# Autodesk Inventor assembly: 三組合窗_MIR2
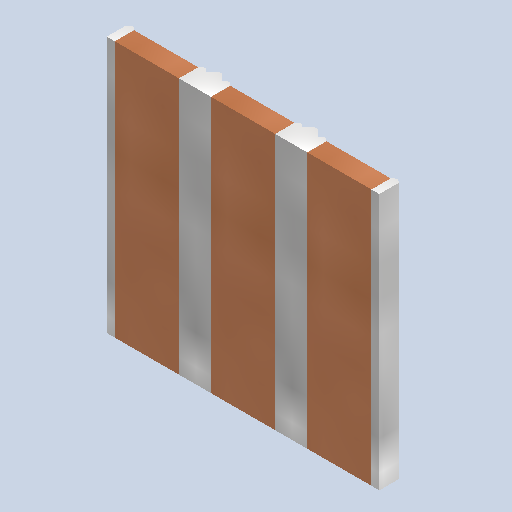
[picture p0: Inventor's stored thumbnail of the model, 512x512]
Saved by Autodesk Inventor 2024.2 (Build 282272000, 272)
## iProperties
Created: 2024-06-02
Part Number: 三組合窗_MIR2
Document SubType Name: Assembly
Designer: User
Author: User
## Documents named in this file (4)
- C:\Users\User\OneDrive - 國立中山大學\桌面\創客基礎\final_project\mirror\三組合窗_MIR2.iam
- C:\Users\User\OneDrive - 國立中山大學\桌面\創客基礎\final_project\mirror\窗_MIR6.ipt
- C:\Users\User\OneDrive - 國立中山大學\桌面\創客基礎\final_project\mirror\窗側柱_MIR6.ipt
- C:\Users\User\OneDrive - 國立中山大學\桌面\創客基礎\final_project\mirror\窗間柱_MIR5.ipt
## Components (7 placed, 3 different names)
1. 窗_MIR6:1 — 齊平:12, 齊平:1, 貼合:6, 齊平:11, 齊平:2, 貼合:2
2. 窗_MIR6:2 — 齊平:9, 齊平:4, 貼合:4, 齊平:10, 齊平:3, 貼合:1
3. 窗_MIR6:3 — 齊平:7, 齊平:6, 貼合:5, 齊平:8, 齊平:5, 貼合:3
4. 窗側柱_MIR6:1 — 齊平:12, 齊平:1, 貼合:6
5. 窗側柱_MIR6:2 — 齊平:7, 齊平:6, 貼合:5
6. 窗間柱_MIR5:1 — 齊平:9, 齊平:8, 齊平:5, 齊平:4, 貼合:4, 貼合:3
7. 窗間柱_MIR5:2 — 齊平:11, 齊平:10, 齊平:3, 齊平:2, 貼合:2, 貼合:1
## Relationships (18: Flush 12, Mate 6)
- 齊平:12 [Flush]: 窗_MIR6:1 ↔ 窗側柱_MIR6:1
- 齊平:1 [Flush]: 窗_MIR6:1 ↔ 窗側柱_MIR6:1
- 貼合:6 [Mate]: 窗_MIR6:1 ↔ 窗側柱_MIR6:1
- 齊平:7 [Flush]: 窗_MIR6:3 ↔ 窗側柱_MIR6:2
- 齊平:6 [Flush]: 窗_MIR6:3 ↔ 窗側柱_MIR6:2
- 貼合:5 [Mate]: 窗_MIR6:3 ↔ 窗側柱_MIR6:2
- 齊平:9 [Flush]: 窗_MIR6:2 ↔ 窗間柱_MIR5:1
- 齊平:8 [Flush]: 窗_MIR6:3 ↔ 窗間柱_MIR5:1
- 齊平:5 [Flush]: 窗_MIR6:3 ↔ 窗間柱_MIR5:1
- 齊平:4 [Flush]: 窗_MIR6:2 ↔ 窗間柱_MIR5:1
- 貼合:4 [Mate]: 窗_MIR6:2 ↔ 窗間柱_MIR5:1
- 貼合:3 [Mate]: 窗_MIR6:3 ↔ 窗間柱_MIR5:1
- 齊平:11 [Flush]: 窗_MIR6:1 ↔ 窗間柱_MIR5:2
- 齊平:10 [Flush]: 窗_MIR6:2 ↔ 窗間柱_MIR5:2
- 齊平:3 [Flush]: 窗_MIR6:2 ↔ 窗間柱_MIR5:2
- 齊平:2 [Flush]: 窗_MIR6:1 ↔ 窗間柱_MIR5:2
- 貼合:2 [Mate]: 窗_MIR6:1 ↔ 窗間柱_MIR5:2
- 貼合:1 [Mate]: 窗_MIR6:2 ↔ 窗間柱_MIR5:2
